# Autodesk Inventor assembly: combination
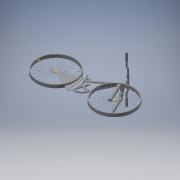
[picture p0: Inventor's stored thumbnail of the model, 180x180]
Saved by Autodesk Inventor 2019 (Build 230136000, 136)
## iProperties
Created: 2021-04-09
Part Number: combination
Material: 一般
Document SubType Name: Assembly
Designer: cadlab
Author: cadlab
## Documents named in this file (10)
- F:\4072pj3\project3\40723102\bike\combination.iam
- F:\4072pj3\project3\40723102\bike\Frame.ipt
- F:\4072pj3\project3\40723102\bike\Triangle fame1.ipt
- F:\4072pj3\project3\40723102\bike\Triangle fame.ipt
- F:\4072pj3\project3\40723102\bike\Slider.ipt
- F:\4072pj3\project3\40723102\bike\Slider1.ipt
- F:\4072pj3\project3\40723102\bike\Rod.ipt
- F:\4072pj3\project3\40723102\bike\Wheel.ipt
- F:\4072pj3\project3\40723102\bike\Handlebar.ipt
- F:\4072pj3\project3\40723102\bike\Fork.ipt
## Components (10 placed, 9 different names)
1. Frame:1 — 貼合:4, 圓柱:2, 貼合:9
2. Triangle fame:1 — 角度:1, 貼合:5, 齊平:4, 貼合:7, 角度:2, 角度:3, 角度:4, 貼合:10
3. Slider:1 — 角度:1, 圓柱:1, 貼合:11, 齊平:6
4. Slider1:1 — 貼合:4, 圓柱:1, 貼合:6
5. Rod:1 — 貼合:5, 貼合:6, 齊平:4
6. Wheel:1 — 貼合:7, 角度:2
7. Wheel:2 — 角度:3, 貼合:8
8. Handlebar:1 — 插入:1
9. Fork:1 — 圓柱:2, 角度:4, 插入:1, 貼合:8
10. Triangle fame1:1 — 貼合:9, 貼合:10, 貼合:11, 齊平:5, 齊平:6
## Relationships (18: Mate 8, Angle 4, Flush 3, CylindricalJoint 2, Insert 1)
- 貼合:4 [Mate]: Frame:1 ↔ Slider1:1
- 角度:1 [Angle] (0 deg): Triangle fame:1 ↔ Slider:1
- 圓柱:1 [CylindricalJoint]: Slider:1 ↔ Slider1:1
- 貼合:5 [Mate]: Triangle fame:1 ↔ Rod:1
- 貼合:6 [Mate]: Slider1:1 ↔ Rod:1
- 齊平:4 [Flush]: Triangle fame:1 ↔ Rod:1
- 貼合:7 [Mate]: Triangle fame:1 ↔ Wheel:1
- 角度:2 [Angle] (0 deg): Triangle fame:1 ↔ Wheel:1
- 角度:3 [Angle] (0 deg): Triangle fame:1 ↔ Wheel:2
- 圓柱:2 [CylindricalJoint]: Frame:1 ↔ Fork:1
- 角度:4 [Angle] (0 deg): Triangle fame:1 ↔ Fork:1
- 插入:1 [Insert]: Handlebar:1 ↔ Fork:1
- 貼合:8 [Mate]: Wheel:2 ↔ Fork:1
- 貼合:9 [Mate]: Frame:1 ↔ Triangle fame1:1
- 貼合:10 [Mate]: Triangle fame:1 ↔ Triangle fame1:1
- 貼合:11 [Mate]: Slider:1 ↔ Triangle fame1:1
- 齊平:5 [Flush]: Triangle fame1:1
- 齊平:6 [Flush]: Slider:1 ↔ Triangle fame1:1
